# Autodesk Inventor assembly: BG002_huenin20_23
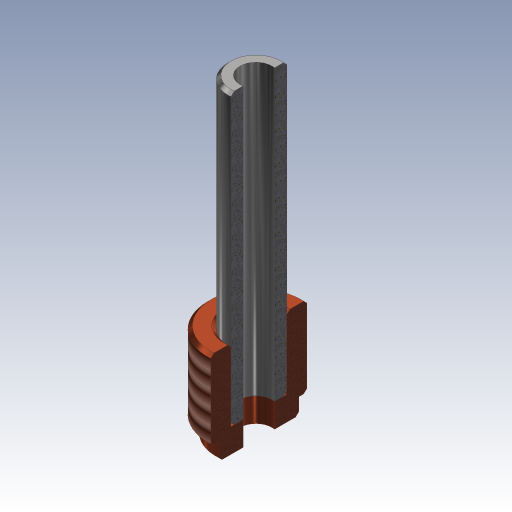
[picture p0: Inventor's stored thumbnail of the model, 512x512]
Saved by Autodesk Inventor 2023.3 (Build 273359000, 359)
## iProperties
Company: HTBLA Kaindorf
RuleStatus: InUse
Created: 2023-08-12
Part Number: BG002_huenin20_23
Project: Fiberprinter-Hotend
Material: Generisch
Description: Heatbreak
Document SubType Name: Assembly
Designer: huenin20
AfterDocNew0: iProperties-Editor_aufrufen
Author: nicob
Keywords: 2023
## Documents named in this file (3)
- C:\Users\nicob\OneDrive\Dokumente\Kop\Fiberprinter_Hotend\BG002_huenin20_23_Fiberprinter-Hotend_Heatbreak.iam
- C:\Users\nicob\OneDrive\Dokumente\Kop\Fiberprinter_Hotend\BT001_huenin20_23_Fiberprinter-Hotend_Heatbreak_thread.ipt
- C:\Users\nicob\OneDrive\Dokumente\Kop\Fiberprinter_Hotend\BT002_huenin20_23_Fiberprinter-Hotend_Heatbreak_pipe.ipt
## Components (2 placed, 2 different names)
1. BT001_huenin20_23_Fiberprinter-Hotend_Heatbreak_thread:1 — Einfügen:1
2. BT002_huenin20_23_Fiberprinter-Hotend_Heatbreak_pipe:1 — Einfügen:1
## Relationships (1: Insert 1)
- Einfügen:1 [Insert]: BT001_huenin20_23_Fiberprinter-Hotend_Heatbreak_thread:1 ↔ BT002_huenin20_23_Fiberprinter-Hotend_Heatbreak_pipe:1
